# Autodesk Inventor assembly: derivado_stokc_resina
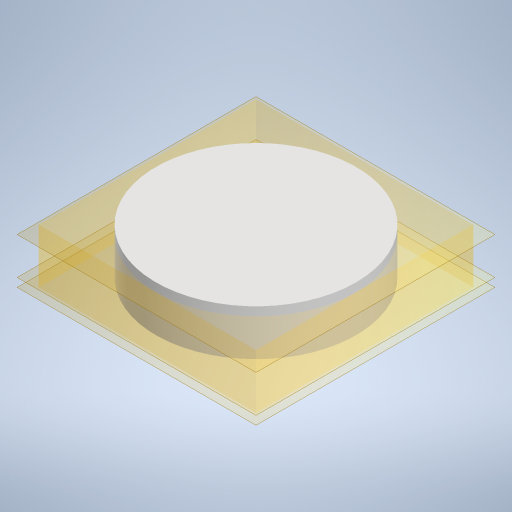
[picture p0: Inventor's stored thumbnail of the model, 512x512]
Saved by Autodesk Inventor 2023.2 (Build 272271030, 271C)
## iProperties
Created: 2023-07-31
Part Number: derivado_stokc_resina
Document SubType Name: Assembly
Designer: Cris Pat
Author: Cris Pat
## Documents named in this file (3)
- C:\Users\Cris Pat\Desktop\U\Semestre_10\Disenio_y_manufactura\proyecto\derivado_stokc_resina.iam
- C:\Users\Cris Pat\Desktop\U\Semestre_10\Disenio_y_manufactura\proyecto\el derivado.ipt
- C:\Users\Cris Pat\Desktop\U\Semestre_10\Disenio_y_manufactura\proyecto\stock material 1.ipt
## Components (2 placed, 2 different names)
1. el derivado:1
2. stock material 1:1 — Flush:1
## Relationships (1: Flush 1)
- Flush:1: stock material 1:1
